# Autodesk Inventor assembly: 041-DP
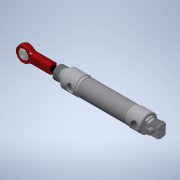
[picture p0: Inventor's stored thumbnail of the model, 180x180]
Saved by Autodesk Inventor 2022.3 (Build 263350000, 350)
## iProperties
Created: 2023-02-26
Part Number: 041-DP
Catalog Web Link: www.cadenas.de
Description: Original Line Standard Air Cylinders-Standard Air Cylinders
Vendor: BIMBA
Document SubType Name: Assembly
Designer: psAdmin
Manufacturer: BIMBA
Mass: 30.4714 g
Surface Area: 196.16 cm^2
Volume: 30.4714 cm^3
Density: 1 g/cm^3
Category: PARTsolutions
Company: BIMBA
PSOL_IDENT_0: {$CADENAS_DATA/23d-libs/bimba/bimba_brand/bimba_imperial/bimba_full_line/original_line_cylinders/sta
PSOL_IDENT_1: ndard_air_cylinders/standard_air_cylinder_asmtab.prj},320 {VTYP=3D},{STYP=ASSTAB},{NB=041-DP},{LINA=
PSOL_IDENT_2: 041-DP},{NN=Original Line Standard Air Cylinders},{DATE=26.01.2023 11:48:58},{GEOMDATE=25.01.2023 07
PSOL_IDENT_3: :23:18},{VERSION=},{LINEID=50},{WBVAR=STROKE,ACTING,MNT,DER,NR,BM,CO,OO,VO,M,EE,EEL,K,Q,Y,G,T,HL,B,H
PSOL_IDENT_4: ,SER,SR,NT,W,STPT1,STPT2,STPT3,STPT4,MB,PB,PRC,TB,MN},{WBNUMERIC=STROKE,EEL}  {NB=041-DP},{LINA=041-
PSOL_IDENT_5: DP},{KT=DUMMY},{PN=041-DP},{PNC=041-DP},{PNA=(NO ACCESSORIES)},{PNAHELP=},{DASH=-},{BORE1=0.75000000
PSOL_IDENT_6: },{BORE=3/4\" (04)},{BOREPN=04},{STROKE=1.000},{STROKEALG=[0.011:50/0.001]},{STROKE1=1.000},{ACTING=
PSOL_IDENT_7: D},{ACTINGALG= '' , 'Single Acting' , 'R' , 'Reverse Single Acting (R)' , 'D' , 'Double Acting (D)'
PSOL_IDENT_8: },{ACTINGPN=D},{MNT=P},{MNTALG= '' , 'Front Nose Mounting' , 'P' , 'Rear Pivot Mounting (P)' , 'XP'
PSOL_IDENT_9: , 'Double End or Pivot Mounting (XP)' , 'X' , 'Double End Mounting (X)' , 'BF' , 'Front Block Mounti
PSOL_IDENT_10: ng (BF)' , 'BR' , 'Rear Block Mounting for Vertical Positioning (BR)' , 'BFT' , 'Front Block Trunnio
PSOL_IDENT_11: n Mounting (BFT)' , 'BRT' , 'Rear Block Trunnion Mounting (BRT)' },{TYPE=},{MNTPN=P},{DER=},{DERALG=
PSOL_IDENT_12: '' , 'N/A' },{NR=},{NRALG= '' , 'N/A' },{NRPN=},{BM=},{BMALG= '' , 'N/A' },{BMPN=},{CO=},{COALG= ''
PSOL_IDENT_13: , 'N/A' },{OO=},{OOALG= '', 'N/A' },{OOPN=},{VO=Z},{VOALG= 'Z' , 'N/A' },{VOPN=},{OOVOPN=},{M=},{MA
PSOL_IDENT_14: LG= '', 'Without Magnet', 'M', 'With Magnet' },{EE=},{EEL=0.000},{EEMAX=49.0000},{EEALG= '', 'Withou
PSOL_IDENT_15: t Extra Extension', 'EE', 'With Extra Extension' },{EELALG=0},{EEPN=},{EEPN1=0.000},{K=},{KALG= '', '
PSOL_IDENT_16: Standard' , 'K' , 'Ports Rotated 90deg K' },{KPN=},{Q=},{QALG= '' , 'N/A' },{QPN=},{Y=},{YALG= '' , '
PSOL_IDENT_17: Without Pivot Bushing' , 'Y' , 'With Pivot Bushing' },{YPN=},{YCON=},{F=},{FALG= '', 'Non-Coated (St
PSOL_IDENT_18: andard)', 'F', 'Molycoated' },{FPN=},{G=},{GPN=},{GPN99=},{T=},{TALG= '' , 'Standard -20° to 200°F (
PSOL_IDENT_19: -29° to 95°C)' , 'N' , 'Low Temperature' , 'V' , 'High Temperature' },{NPN=},{VPN=},{HL=},{HLALG= ''
PSOL_IDENT_20: , 'Without Low Pressure Hydraulic' , 'HL' , 'With Low Pressure Hydraulic' },{B=},{BALG= '', 'W/out
PSOL_IDENT_21: Bumpers' , 'B' , 'W/ Bumpers' },{BPN=},{H=},{HALG= '', 'N/A' },{HPN=},{SER=},{SERALG= '' , 'Without
PSOL_IDENT_22: Spring Extend/Return' , 'JS' , 'With Spring Return' , 'JR' , 'With Spring Extend' },{SR=C},{SRALG= '
PSOL_IDENT_23: C' , 'Standard Blackened Carbon Steel' , 'SR' , 'Stainless Steel [SR]' },{SRPN=},{SRCON=1},{NT=},{NT
PSOL_IDENT_24: PN=},{W=},{WALG= '' , 'Without Wiper' , 'W' , 'With Wiper' },{WPN=},{E=},{EALG= '' , 'Standard Seals
PSOL_IDENT_25: /Lube' , 'E' , 'Non-Lube Seals/Lube' },{EPN=},{ST=},{STALG= '' , 'N/A' },{STPT1=},{STPT1ALG= '' , 'N
PSOL_IDENT_26: /A' },{STPT2=},{STPT2ALG= '' , 'N/A' },{STPT3=},{STPT3ALG= '' , 'N/A' },{STPT4=},{STPT4ALG= '' , 'N/
PSOL_IDENT_27: A' },{STPN=},{MB=},{MBALG= '' , 'N/A' },{MBPN=},{MBPNALL=},{MBPNALLREAR=},{PB=},{PBALG= '' , 'Withou
PSOL_IDENT_28: t Pivot Bracket' , 'D-167' , 'D-167' },{PBPN=},{PBPNALL=D-167},{PRC=},{PRCALG= '' , 'W/out Pivot Rod
PSOL_IDENT_29: Clevis' , 'F,D-166-3' , 'D-166-3 (front)' },{PRCPN=},{PRCPNALL=D-166-3},{TB=},{TBALG= '' , 'N/A' },
PSOL_IDENT_30: {TBPN=},{TBPNALL=},{MN=},{MNALG= '' , 'Without Mounting Nut' , 'F,D-9' , 'D-9 (front)' , 'R,D-9' , '
PSOL_IDENT_31: D-9 (rear)', '2x,D-9' , 'D-9 (front & rear)' },{MNPN=},{MNCONF=},{MNCONR=},{TLEN=2.2555},{FRAC=4.750
PSOL_IDENT_32: 0},{RGCON=},{RGDACCON=R},{RHCON=P},{RHCON1=P},{RHCONON=1},{RHACCON=},{FNUTCON=0},{RNUTCON=0},{FNUTPN=
PSOL_IDENT_33: D-9},{RNUTPN=D-9},{FNUTTRANS=0.0000},{RNUTTRANS=0.0000},{VHOLECON=0},{A1=1.5940},{A1N=0.8750},{A1P=1
PSOL_IDENT_34: .5940},{A1B=1.5940},{A4=0.2525},{A4N=0.3130},{A4P=0.2525},{A5=0.0300},{A1H=1.594},{A1NH=0.5310},{A1P
PSOL_IDENT_35: H=1.5940},{A1BH=1.0940},{A1SH=1.2190},{A2H=0.2190},{A2NH=0.2190},{LENGTH=3.7500},{LENGTH1=3.7500},{L
PSOL_IDENT_36: ENGTH2=3.8100},{MUL=1.0000},{MUL11=1.0000},{MUL22=2.69},{MUL33=1.6900},{MUL2=1.0000},{MUL211=1.0000}
PSOL_IDENT_37: ,{MUL222=2.6900},{MUL233=1.6900},{SSS=2.0000},{RGLEN=1.3715},{RHLEN=1.1230},{SSS1=2.0000},{A13=1.312
PSOL_IDENT_38: 0},{DIF=0.0000},{G5=0.6250},{ON=0},{SSADD=0.0000},{BADD=0.0000},{MADD=0.0000},{NVADD=0.0000},{TRACKL=
PSOL_IDENT_39: 1.9655},{TRACKCON=D-74168},{TRIMCON=0},{TRIMCON1=0},{PINCON=D-51},{FSPACE=0.5234},{SPACE=0.0536},{TE
PSOL_IDENT_40: XT=0.0938},{S1=1.0000},{D1=0.8325},{D1N=0.8050},{D1B=0.8625},{D1P=0.8325},{FA=0.940},{RA=0.9400},{PP
PSOL_IDENT_41: ATH=standard_air_cylinder_asmtpl.prj},{MATALGHTML=<b>Standard Original Line:</b><dl><dt>Rod:</dt><dd
PSOL_IDENT_42: >- Stainless Steel</dd><dd>&nbsp;&nbsp;(5/16 9/16 Bores)</dd><dd>- High Strength Carbon Steel</dd><d
PSOL_IDENT_43: d>&nbsp;&nbsp;(3/4 3 Bore)</dd><dd>- Stainless Steel</dd><dd>&nbsp;&nbsp;(X style DXP/DX/DXDE)</dd><
PSOL_IDENT_44: dt>Bearings:</dt><dd>- Sintered Bronze</dd><dt>Body:</dt><dd>- 304 Stainless Steel</dd><dt>End Caps:
PSOL_IDENT_45: </dt><dd>- Aluminum</dd><dt>Seals:</dt><dd>- Buna N</dd></dl>},{ASSCFGPRA=04DP},{MBPNA=},{MNPNA=},{P
PSOL_IDENT_46: RCPNA=},{ASSOPTACC=STPT4},{A=4.75},{HADD=0.0000},{WFL=0.25},{QADD=0.000},{QADD1=0.440},{TEST=1.0000}
PSOL_IDENT_47: ,{MNTB=},{STDNUTF=0},{STDNUTR=0},{STRK2D=0},{X2D=2},{STROKESW=1.000},{EESW=0.000},{FCD=0},{BCD=0},{R
PSOL_IDENT_48: CD=0},{CUSTADD=0.000},{FT=1/4-28 UNF-2A},{FT1=1/4-28 UNF-2A},{FT2=5/8-18 UNF-2A},{PORT=1/8 NPT},{POR
PSOL_IDENT_49: T1=1/8 NPT},{PORT2=1/8 NPT},{FT11=1/2-20 UNF-2A},{FT12=5/8-18 UNF-2A},{B1=}
NB: 041-DP
NN: Original Line Standard Air Cylinders
NT: Threaded (Standard)
NBSYN: $PNC.
LINA: 041-DP
CATALOG: Bimba Products
PN: 041-DP
PNA: (NO ACCESSORIES)
BORE: 3/4" (04)
STROKE: 1
ACTING: Double Acting (D)
MNT: Rear Pivot Mounting (P)
DER: N/A
NR: N/A
CO: N/A
OO: N/A
VO: N/A
M: Without Magnet
EE: Without Extra Extension
EEL: 0
K: Standard
Q: N/A
Y: Without Pivot Bushing
G: Standard Lube
T: Standard -20° to 200°F (-29° to 95°C)
HL: Without Low Pressure Hydraulic
B: W/out Bumpers
H: N/A
SER: Without Spring Extend/Return
SR: Standard Blackened Carbon Steel
W: Without Wiper
STPT1: N/A
STPT2: N/A
STPT3: N/A
STPT4: N/A
MB: N/A
PB: Without Pivot Bracket
PRC: W/out Pivot Rod Clevis
TB: N/A
MN: Without Mounting Nut
A: 4.75
SUPPLIER: BIMBA
ARTICLENO: 041-DP
BOMINFO: 041-DP
CREATOR: CADENAS GmbH
Title: 041-DP
Author: Cadenas PARTsolutions
Comments: Standard Air Cylinders
## Documents named in this file (8)
- C:\Users\mavericks\Desktop\2023-Charged-Up\COMMON PARTS\AIR CYLINDERS\BIMBA_041DP\AIS2022\041-DP.iam
- C:\Users\mavericks\Desktop\2023-Charged-Up\COMMON PARTS\AIR CYLINDERS\BIMBA_041DP\AIS2022\041-DPC0000000_0_dummy.ipt
- C:\Users\mavericks\Desktop\2023-Charged-Up\COMMON PARTS\AIR CYLINDERS\BIMBA_041DP\AIS2022\04R000-0_rod_guide.ipt
- C:\Users\mavericks\Desktop\2023-Charged-Up\COMMON PARTS\AIR CYLINDERS\BIMBA_041DP\AIS2022\04R-2_25550C.ipt
- C:\Users\mavericks\Desktop\2023-Charged-Up\COMMON PARTS\AIR CYLINDERS\BIMBA_041DP\AIS2022\04P0000_rear_head.ipt
- C:\Users\mavericks\Desktop\2023-Charged-Up\COMMON PARTS\AIR CYLINDERS\BIMBA_041DP\AIS2022\D-51.ipt
- C:\Users\mavericks\Desktop\2023-Charged-Up\COMMON PARTS\AIR CYLINDERS\BIMBA_041DP\AIS2022\C-041-DP0000_rod.ipt
- C:\Users\mavericks\Desktop\2023-Charged-Up\COMMON PARTS\AIR CYLINDERS\TieRod End\60685K321_PTFE-LINED ALUMINUM BALL JOINT ROD END.ipt
## Components (7 placed, 7 different names)
1. 041-DPC0000000_0_dummy:1
2. 04R000-0_rod_guide:1 — Insert:1
3. 04R-2_25550C:1
4. 04P0000_rear_head:1 — Angle:1
5. D-51:1
6. C-041-DP0000_rod:1 — Insert:1, Insert:2
7. 60685K321_PTFE-LINED ALUMINUM BALL JOINT ROD END:1 — Insert:2, Angle:1
## Relationships (3: Insert 2, Angle 1)
- Insert:1: 04R000-0_rod_guide:1 ↔ C-041-DP0000_rod:1
- Insert:2 (6.35 mm): C-041-DP0000_rod:1 ↔ 60685K321_PTFE-LINED ALUMINUM BALL JOINT ROD END:1
- Angle:1 (0 deg): 04P0000_rear_head:1 ↔ 60685K321_PTFE-LINED ALUMINUM BALL JOINT ROD END:1
